# Autodesk Inventor assembly: copy_stand
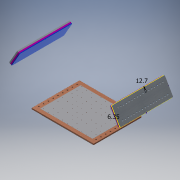
[picture p0: Inventor's stored thumbnail of the model, 180x180]
Saved by Autodesk Inventor 2019 (Build 230136000, 136)
## iProperties
Created: 2018-12-01
Part Number: copy_stand
Document SubType Name: Assembly
Designer: caleb
Author: caleb
## Documents named in this file (7)
- C:\cygwin64\home\caleb\copy_stand\copy_stand.iam
- C:\cygwin64\home\caleb\copy_stand\copy_stand_light.ipt
- C:\cygwin64\home\caleb\copy_stand\paper.ipt
- C:\cygwin64\home\caleb\copy_stand\copy_stand_base.ipt
- C:\cygwin64\home\caleb\copy_stand\copy_stand_light_MIR.ipt
- C:\cygwin64\home\caleb\copy_stand\copy_stand_light.iam
- C:\Users\caleb\Documents\Inventor\Content Center Files\R2019\en-US\ANSI B18.6.3(25)\ANSI B18.6.3 - 1_4-28 UNF - 0.375(5).ipt
## Components (6 placed, 5 different names)
1. copy_stand_light:1 — Mate:1, Mate:2, Angle:1, Mate:4
2. paper:1 — Flush:1, Mate:3, Flush:2
3. copy_stand_base:1 — Flush:1, Mate:1, Mate:2, Mate:3, Flush:2, Angle:1
4. copy_stand_light_MIR:1
5. copy_stand_light:2 [sub-assembly]
6. Cross Recessed Pan Head Machine Screw - Type IA - Inch 1/4 - 28 - 3/8:1 — Mate:4
## Relationships (7: Mate 4, Flush 2, Angle 1)
- Flush:1: paper:1 ↔ copy_stand_base:1
- Mate:1: copy_stand_light:1 ↔ copy_stand_base:1
- Mate:2 (152.4 mm): copy_stand_light:1 ↔ copy_stand_base:1
- Mate:3: paper:1 ↔ copy_stand_base:1
- Flush:2: paper:1 ↔ copy_stand_base:1
- Angle:1 (120 deg): copy_stand_light:1 ↔ copy_stand_base:1
- Mate:4: copy_stand_light:1 ↔ Cross Recessed Pan Head Machine Screw - Type IA - Inch 1/4 - 28 - 3/8:1
